# Autodesk Inventor assembly: CL-4-F
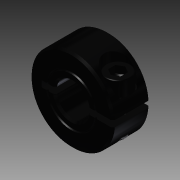
[picture p0: Inventor's stored thumbnail of the model, 180x180]
Saved by Autodesk Inventor 2014 (Build 180170000, 170)
## iProperties
Category: Miscellaneous
Company: Autodesk Inc.
Created: 2013-12-18
Part Number: CL-4-F
Document SubType Name: Assembly
Designer: Autodesk Inc.
Catalog Web Link: http://www.ruland.com/shaft-collar.php?recordID=CL-4-F
Description: 1/4 " ID 1/2" OD Clamp Shaft Collar
Vendor: Ruland Manufacturing
Author: Autodesk Inc.
## Documents named in this file (3)
- D:\Data Folder\FIRST 2014\KOP Parts\Miscellaneous\MISC_ShaftCollar_CL-4-F.iam
- D:\Data Folder\FIRST 2014\KOP Parts\Miscellaneous\MISC_ShaftCollar_CL-4-F.ipt
- D:\Data Folder\FIRST 2014\KOP Parts\Miscellaneous\ANSI B18.3 - 4-40 UNC - 0.3125(31).ipt
## Components (2 placed, 2 different names)
1. MISC_ShaftCollar_CL-4-F:1 — Insert:1
2. Hexagon Socket Head Cap Screw - Inch No. 4 - 40 UNC - 5/16:1 — Insert:1
## Relationships (1: Insert 1)
- Insert:1: MISC_ShaftCollar_CL-4-F:1 ↔ Hexagon Socket Head Cap Screw - Inch No. 4 - 40 UNC - 5/16:1
